# Autodesk Inventor assembly: nicuneck
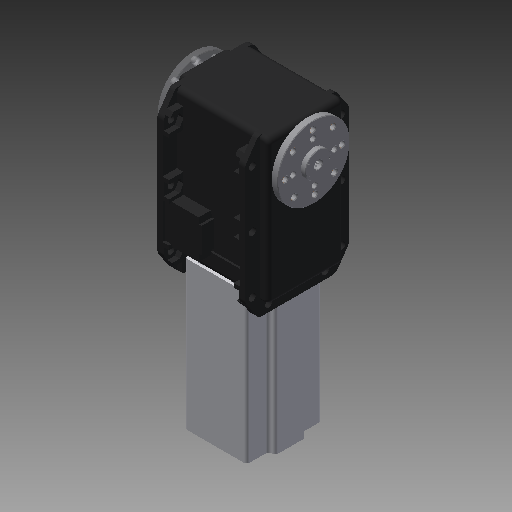
[picture p0: Inventor's stored thumbnail of the model, 512x512]
Saved by Autodesk Inventor 2019 (Build 230136000, 136)
## iProperties
Created: 2015-02-23
Part Number: nicuneck
Document SubType Name: Assembly
Designer: 4mahboob
Mass: 90.4387 g
Surface Area: 242.156 cm^2
Volume: 90.4387 cm^3
Density: 1 g/cm^3
Author: 4mahboob
## Documents named in this file (3)
- Z:\Nico_N\NICO-CAD-master\NICO_CAD_master\head\neck.iam
- Z:\Nico_N\NICO-CAD-master\NICO_CAD_master\head\headnickholder_long.ipt
- Z:\Nico_N\NICO-CAD-master\NICO_CAD_master\motors\Mx64\Mx64_with_horn_and_bearing.iam
## Components (2 placed, 2 different names)
1. headnickholder_long:1 — Insert:1, Insert:2
2. Mx64_with_horn_and_bearing:1 [sub-assembly] — Insert:1, Insert:2
## Relationships (2: Insert 2)
- Insert:1 (2.5 mm): headnickholder_long:1 ↔ Mx64_with_horn_and_bearing:1
- Insert:2 (2.5 mm): headnickholder_long:1 ↔ Mx64_with_horn_and_bearing:1
